# Autodesk Inventor assembly: Capping_Assembly2
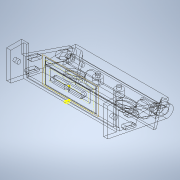
[picture p0: Inventor's stored thumbnail of the model, 180x180]
Saved by Autodesk Inventor 2022 (Build 260153000, 153)
## iProperties
Created: 2024-05-05
Part Number: Capping_Assembly2
Document SubType Name: Assembly
Designer: raphael.hauk
Author: raphael.hauk
## iProperties of the stored document Holder - Printheadfixture.ipt
Created: 2024-05-05
Part Number: Holder - Printheadfixture
Material: Generic
Description: STEP AP242
Document SubType Name: Modeling
Designer: raphael.hauk
Density: 1 g/cm^3
Appearance: Default
Preprocessor: ST-DEVELOPER v20
Title: 66377de951769f1adeb82ab8
## Documents named in this file (9)
- C:\git\inkjet-printer\cad\Capping_Assembly2.iam
- C:\git\inkjet-printer\cad\Xaar128.ipt
- **C:\git\inkjet-printer\cad\Capping_Assembly2.iam*LocalDocs*xAaaaq0aaAaaaaaaaAaaaq4fc4g*Holder - Printheadfixture.ipt
- C:\git\inkjet-printer\cad\Capping_Insert.ipt
- C:\git\inkjet-printer\cad\Capping_RotationAnchor.ipt
- C:\git\inkjet-printer\cad\Capping_RotatingCover.ipt
- C:\git\inkjet-printer\cad\Capping_RotatingArm.ipt
- C:\git\inkjet-printer\cad\Capping_RubberInsert.ipt
- C:\git\inkjet-printer\cad\Holder - Printheadfixture.step
## Components (7 placed, 7 different names)
1. Xaar128:1 — Mate:1, Mate:2, Rotational:1, Rotational:2, Flush:1, Mate:4, Angle:1, Angle:2, Flush:12
2. Holder - Printheadfixture:1 — Mate:2, Rotational:1, Rotational:2, Flush:3
3. Capping_Insert:1 — Flush:1, Mate:4, Flush:9, Mate:5, Mate:6, Mate:7
4. Capping_RotationAnchor:1 — Flush:2, Flush:3, Flush:9
5. Capping_RotatingCover:1 — Mate:5, Mate:6, Mate:7, Mate:8, Flush:11
6. Capping_RotatingArm:1 — Mate:8, Flush:11
7. Capping_RubberInsert:1 — Flush:12
## Relationships (17: Mate 7, Flush 6, RevoluteJoint 2, Angle 2)
- Mate:1: Xaar128:1
- Mate:2: Xaar128:1 ↔ Holder - Printheadfixture:1
- Rotational:1 [RevoluteJoint]: Xaar128:1 ↔ Holder - Printheadfixture:1
- Rotational:2 [RevoluteJoint]: Xaar128:1 ↔ Holder - Printheadfixture:1
- Flush:1: Xaar128:1 ↔ Capping_Insert:1
- Mate:4: Xaar128:1 ↔ Capping_Insert:1
- Angle:1 (180 deg): Xaar128:1
- Angle:2 (180 deg): Xaar128:1
- Flush:2: Capping_RotationAnchor:1
- Flush:3: Holder - Printheadfixture:1 ↔ Capping_RotationAnchor:1
- Flush:9: Capping_Insert:1 ↔ Capping_RotationAnchor:1
- Mate:5: Capping_Insert:1 ↔ Capping_RotatingCover:1
- Mate:6: Capping_Insert:1 ↔ Capping_RotatingCover:1
- Mate:7 (-0.1 mm): Capping_Insert:1 ↔ Capping_RotatingCover:1
- Mate:8: Capping_RotatingCover:1 ↔ Capping_RotatingArm:1
- Flush:11: Capping_RotatingCover:1 ↔ Capping_RotatingArm:1
- Flush:12: Xaar128:1 ↔ Capping_RubberInsert:1
